# Autodesk Inventor assembly: ensamble_herramienta
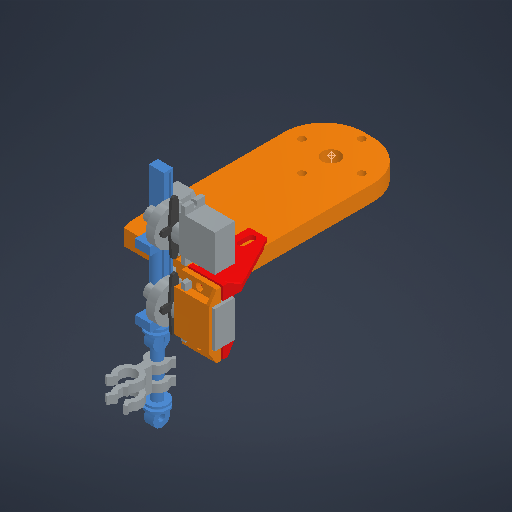
[picture p0: Inventor's stored thumbnail of the model, 512x512]
Saved by Autodesk Inventor 2026.2 (Build 302298000, 298)
## iProperties
Created: 2026-03-12
Part Number: ensamble_herramienta
Document SubType Name: Assembly
Designer: User
Author: User
## Documents named in this file (5)
- E:\Proyectos\scara-robot-rrp\mechanical\inventor\ensamble_herramienta.iam
- E:\Proyectos\scara-robot-rrp\mechanical\inventor\lamina_herrAMIENTA.ipt
- E:\Proyectos\scara-robot-rrp\mechanical\inventor\pinza.iam
- E:\Proyectos\scara-robot-rrp\mechanical\inventor\soporte-motor.ipt
- E:\Proyectos\scara-robot-rrp\mechanical\inventor\soprte_motor.ipt
## Components (4 placed, 4 different names)
1. lamina_herrAMIENTA:1 — Mate:1, Flush:1, Flush:2, Mate:6, Mate:7
2. pinza:1 [sub-assembly] — Mate:1, Flush:1, Flush:2, Mate:2, Mate:3, Mate:4, Mate:5
3. soporte-motor:1 — Mate:4, Flush:4, Flush:5
4. soprte_motor:1 — Mate:2, Mate:3, Flush:4, Flush:5, Mate:5
## Relationships (12: Mate 8, Flush 4)
- Mate:1: lamina_herrAMIENTA:1 ↔ pinza:1
- Flush:1 (12.862 mm): lamina_herrAMIENTA:1 ↔ pinza:1
- Flush:2 (9.5 mm): lamina_herrAMIENTA:1 ↔ pinza:1
- Mate:2: pinza:1 ↔ soprte_motor:1
- Mate:3: pinza:1 ↔ soprte_motor:1
- Mate:4: pinza:1 ↔ soporte-motor:1
- Flush:4: soporte-motor:1 ↔ soprte_motor:1
- Flush:5: soporte-motor:1 ↔ soprte_motor:1
- Mate:5: pinza:1 ↔ soprte_motor:1
- Mate:6: lamina_herrAMIENTA:1
- Mate:7: lamina_herrAMIENTA:1
- Mate:8
